# Autodesk Inventor assembly: Roller Carouel Assembly
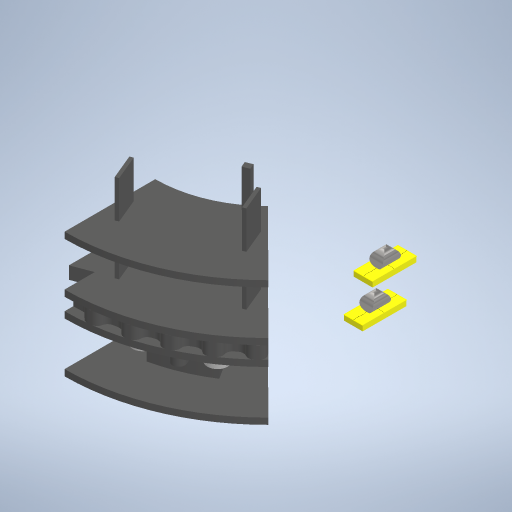
[picture p0: Inventor's stored thumbnail of the model, 512x512]
Saved by Autodesk Inventor 2023 (Build 270158000, 158)
## iProperties
Created: 2022-11-09
Part Number: Roller Carouel Assembly
Document SubType Name: Assembly
Designer: cheng
Mass: 2238.02 g
Surface Area: 4892.44 cm^2
Volume: 2375.07 cm^3
Density: 0.942297 g/cm^3
Author: cheng
## Documents named in this file (6)
- C:\Users\mihal\Desktop\4th Year Project\BHSS DESIGN\Sixth Assembly\Roller Carouel Assembly.iam
- C:\Users\mihal\Desktop\4th Year Project\BHSS DESIGN\Sixth Assembly\Roller Carousel Part.ipt
- C:\Users\mihal\Desktop\4th Year Project\BHSS DESIGN\Sixth Assembly\6002-z-bnl v1.ipt
- C:\Users\mihal\Desktop\4th Year Project\BHSS DESIGN\Sixth Assembly\Carousel Container Plate.ipt
- C:\Users\mihal\Desktop\4th Year Project\BHSS DESIGN\Sixth Assembly\Roller Carousel Gear.ipt
- C:\Users\mihal\Desktop\4th Year Project\BHSS DESIGN\Sixth Assembly\Ball Transfer Unit Assembly.iam
## Components (9 placed, 5 different names)
1. Roller Carousel Part:1 — Rotational:1, Rotational:2, Rotational:3, Rotational:4, Mate:7, Mate:8, Mate:9
2. 6002-z-bnl v1:1 — Rotational:3
3. 6002-z-bnl v1:2 — Rotational:1
4. 6002-z-bnl v1:3 — Rotational:4
5. 6002-z-bnl v1:4 — Rotational:2
6. Carousel Container Plate:1 — Mate:10, Mate:11, Mate:12
7. Roller Carousel Gear:1 — Mate:7, Mate:8, Mate:9, Mate:10, Mate:11, Mate:12
8. Ball Transfer Unit Assembly:1 [sub-assembly]
9. Ball Transfer Unit Assembly:2 [sub-assembly]
## Relationships (10: Mate 6, RevoluteJoint 4)
- Rotational:1 [RevoluteJoint]: Roller Carousel Part:1 ↔ 6002-z-bnl v1:2
- Rotational:2 [RevoluteJoint]: Roller Carousel Part:1 ↔ 6002-z-bnl v1:4
- Rotational:3 [RevoluteJoint]: Roller Carousel Part:1 ↔ 6002-z-bnl v1:1
- Rotational:4 [RevoluteJoint]: Roller Carousel Part:1 ↔ 6002-z-bnl v1:3
- Mate:7: Roller Carousel Part:1 ↔ Roller Carousel Gear:1
- Mate:8: Roller Carousel Part:1 ↔ Roller Carousel Gear:1
- Mate:9: Roller Carousel Part:1 ↔ Roller Carousel Gear:1
- Mate:10: Carousel Container Plate:1 ↔ Roller Carousel Gear:1
- Mate:11: Carousel Container Plate:1 ↔ Roller Carousel Gear:1
- Mate:12: Carousel Container Plate:1 ↔ Roller Carousel Gear:1
